# Autodesk Inventor assembly: Assembly2
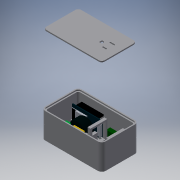
[picture p0: Inventor's stored thumbnail of the model, 180x180]
Saved by Autodesk Inventor 2019 (Build 230136000, 136)
## iProperties
Created: 2022-02-04
Part Number: Assembly2
Document SubType Name: Assembly
Designer: josec
Author: josec
## Documents named in this file (9)
- C:\Users\josec\Documents\Inventor\Enchufe\Assembly2.iam
- C:\Users\josec\Documents\Inventor\Enchufe\base2.ipt
- C:\Users\josec\Documents\Inventor\Enchufe\PZEM-00ET.ipt
- C:\Users\josec\Documents\Inventor\Enchufe\ESP32.ipt
- C:\Users\josec\Documents\Inventor\Enchufe\power supply2.ipt
- C:\Users\josec\Documents\Inventor\Enchufe\coil.ipt
- C:\Users\josec\Documents\Inventor\Enchufe\sop.ipt
- C:\Users\josec\Documents\Inventor\Enchufe\cover.ipt
- C:\Users\josec\Documents\Inventor\Enchufe\top.ipt
## Components (10 placed, 8 different names)
1. base2:1 — Mate:1, Mate:2, Mate:3, Mate:4, Mate:5, Flush:1, Mate:6, Mate:7, Mate:8, Rotational:1, Mate:9, Flush:2, Flush:3, Mate:10, Flush:4, Flush:5, Mate:11, Mate:12, Mate:13
2. PZEM-00ET:1 — Mate:1, Mate:2, Mate:3
3. power supply2:3 — Mate:4, Mate:5, Flush:1
4. ESP32:1 — Mate:6, Mate:7, Mate:8
5. coil:1 — Rotational:1
6. sop:1 — Mate:9, Flush:2, Flush:3
7. sop:2 — Mate:10, Flush:4, Flush:5
8. cover:1 — Mate:11, Mate:12, Mate:13, Mate:14, Flush:6, Flush:7
9. cover:2 — Mate:14, Flush:6, Flush:7, Mate:15, Mate:16
10. top:1 — Mate:15, Mate:16
## Relationships (24: Mate 16, Flush 7, RevoluteJoint 1)
- Mate:1: base2:1 ↔ PZEM-00ET:1
- Mate:2: base2:1 ↔ PZEM-00ET:1
- Mate:3: base2:1 ↔ PZEM-00ET:1
- Mate:4: base2:1 ↔ power supply2:3
- Mate:5: base2:1 ↔ power supply2:3
- Flush:1: base2:1 ↔ power supply2:3
- Mate:6: base2:1 ↔ ESP32:1
- Mate:7: base2:1 ↔ ESP32:1
- Mate:8: base2:1 ↔ ESP32:1
- Rotational:1 [RevoluteJoint]: base2:1 ↔ coil:1
- Mate:9: base2:1 ↔ sop:1
- Flush:2: base2:1 ↔ sop:1
- Flush:3: base2:1 ↔ sop:1
- Mate:10: base2:1 ↔ sop:2
- Flush:4: base2:1 ↔ sop:2
- Flush:5: base2:1 ↔ sop:2
- Mate:11: base2:1 ↔ cover:1
- Mate:12: base2:1 ↔ cover:1
- Mate:13: base2:1 ↔ cover:1
- Mate:14: cover:1 ↔ cover:2
- Flush:6: cover:1 ↔ cover:2
- Flush:7: cover:1 ↔ cover:2
- Mate:15: cover:2 ↔ top:1
- Mate:16: cover:2 ↔ top:1
